# Autodesk Inventor assembly: 310-2
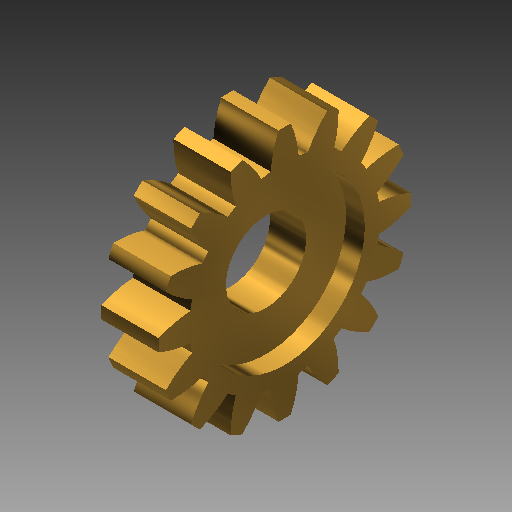
[picture p0: Inventor's stored thumbnail of the model, 512x512]
Saved by Autodesk Inventor 2019 (Build 230136000, 136)
## iProperties
Company: Autodesk Inc.
Created: 2017-05-31
Part Number: 310-2
Document SubType Name: Assembly
Designer: Autodesk Inc.
Mass: 0.739695 g
Surface Area: 2.36864 cm^2
Volume: 0.0873311 cm^3
Density: 8.47 g/cm^3
Author: Inventor
## Documents named in this file (3)
- C:\TEMP\Fishing Rod\Workspaces\Back Drive Transfer Gear.iam
- C:\TEMP\Fishing Rod\Workspaces\Back Drive Transfer Gear\Design Accelerator\Back Drive Transfer Shaft.iam
- C:\TEMP\Fishing Rod\Workspaces\Back Drive Transfer Gear\Design Accelerator\Back Drive Transfer Spur.iam
## Components (2 placed, 2 different names)
1. Shaft:1 [sub-assembly] — Mate:1, Mate:2, Flush:1
2. Spur Gears:1 [sub-assembly]
## Relationships (3: Mate 2, Flush 1)
- Mate:1: Shaft:1
- Mate:2: Shaft:1
- Flush:1: Shaft:1
